# Autodesk Inventor assembly: ZespolDuzegoKola
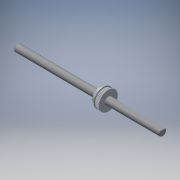
[picture p0: Inventor's stored thumbnail of the model, 180x180]
Saved by Autodesk Inventor 2019.4 (Build 234330000, 330)
## iProperties
Created: 2020-05-23
Part Number: ZespolDuzegoKola
Document SubType Name: Assembly
Designer: estee
Author: estee
## Documents named in this file (4)
- F:\MUM\Od Esterki\ModulDuzegoKola.iam
- F:\MUM\Od Esterki\ISO 4029 - M3 x 6 - ISO.ipt
- F:\MUM\Od Esterki\GT2_50teeth.ipt
- F:\MUM\Od Esterki\walek.ipt
## Components (4 placed, 3 different names)
1. ISO 4029 M3 x 6:1 — Mate:2, Flush:1, Tangent:2
2. ISO 4029 M3 x 6:2 — Mate:3, Tangent:1
3. GT2_50teeth:1 — Mate:1, Mate:2, Mate:3
4. walek:1 — Mate:1, Tangent:1, Flush:1, Tangent:2
## Relationships (6: Mate 3, Tangent 2, Flush 1)
- Mate:1: GT2_50teeth:1 ↔ walek:1
- Mate:2: ISO 4029 M3 x 6:1 ↔ GT2_50teeth:1
- Mate:3: ISO 4029 M3 x 6:2 ↔ GT2_50teeth:1
- Tangent:1 (-18 mm): ISO 4029 M3 x 6:2 ↔ walek:1
- Flush:1 (6 mm): ISO 4029 M3 x 6:1 ↔ walek:1
- Tangent:2: ISO 4029 M3 x 6:1 ↔ walek:1
